# Autodesk Inventor assembly: bluetooth_box
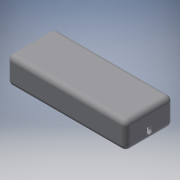
[picture p0: Inventor's stored thumbnail of the model, 180x180]
Saved by Autodesk Inventor 2017 (Build 210142000, 142)
## iProperties
Created: 2017-09-23
Part Number: bluetooth_box
Document SubType Name: Assembly
Designer: Mitch
Author: Mitch
## Documents named in this file (3)
- E:\Youtube Channel\Pojects\Bluetooth Aux\bluetooth_box.iam
- E:\Youtube Channel\Pojects\Bluetooth Aux\box_bottom.ipt
- E:\Youtube Channel\Pojects\Bluetooth Aux\box_top.ipt
## Components (2 placed, 2 different names)
1. box_bottom:1 — Mate:1, Flush:1, Flush:2
2. box_top:1 — Mate:1, Flush:1, Flush:2
## Relationships (3: Flush 2, Mate 1)
- Mate:1: box_bottom:1 ↔ box_top:1
- Flush:1: box_bottom:1 ↔ box_top:1
- Flush:2: box_bottom:1 ↔ box_top:1
